# Autodesk Inventor assembly: шестерни изменяемая траектория
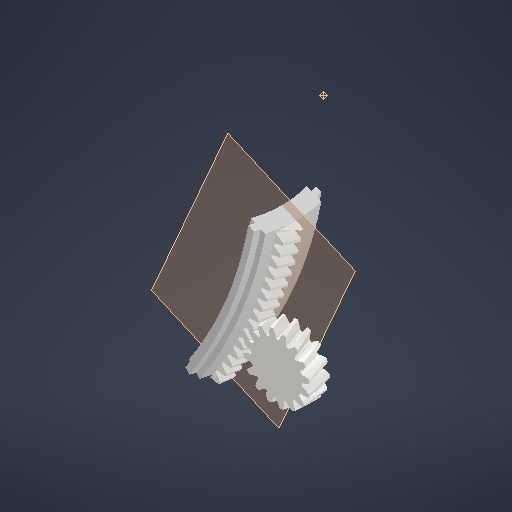
[picture p0: Inventor's stored thumbnail of the model, 512x512]
Saved by Autodesk Inventor 2026.2 (Build 302298000, 298)
## iProperties
Created: 2025-12-06
Part Number: шестерни изменяемая траектория
Document SubType Name: Assembly
Designer: Phantom
Author: Phantom
## Documents named in this file (5)
- C:\Users\Phantom\Desktop\Phantom16950\шестерни изменяемая траектория.iam
- C:\Users\Phantom\Desktop\Phantom16950\шестерни изменяемая траектория\Мастер проектирования\Цилиндрическое зубчатое зацепление2.iam
- C:\Users\Phantom\Desktop\Phantom16950\изменяемая траектория.ipt
- C:\Users\Phantom\Desktop\Phantom16950\пол шестерни для траектории.ipt
- C:\Users\Phantom\Desktop\Phantom16950\пол шестерни мал для траектории.ipt
## Components (4 placed, 4 different names)
1. Цилиндрическое зубчатое зацепление:2 [sub-assembly] — Совмещение:1, Совмещение:5
2. изменяемая траектория:1 — Совмещение:1, Совмещение:5, Совмещение:6, Совмещение:7, Совмещение:8
3. Цилиндрическое зубчатое зацепление2:1 — Совмещение:6, Совмещение:7, Совмещение:8, Совмещение:9, Заподлицо:1
4. Цилиндрическое зубчатое зацепление1:1 — Совмещение:9, Заподлицо:1
## Relationships (7: Mate 6, Flush 1)
- Совмещение:1 [Mate]: Цилиндрическое зубчатое зацепление:2 ↔ изменяемая траектория:1
- Совмещение:5 [Mate]: Цилиндрическое зубчатое зацепление:2 ↔ изменяемая траектория:1
- Совмещение:6 [Mate]: изменяемая траектория:1 ↔ Цилиндрическое зубчатое зацепление2:1
- Совмещение:7 [Mate]: изменяемая траектория:1 ↔ Цилиндрическое зубчатое зацепление2:1
- Совмещение:8 [Mate]: изменяемая траектория:1 ↔ Цилиндрическое зубчатое зацепление2:1
- Совмещение:9 [Mate] (240.643 mm): Цилиндрическое зубчатое зацепление2:1 ↔ Цилиндрическое зубчатое зацепление1:1
- Заподлицо:1 [Flush]: Цилиндрическое зубчатое зацепление2:1 ↔ Цилиндрическое зубчатое зацепление1:1
